# Autodesk Inventor assembly: LF_2
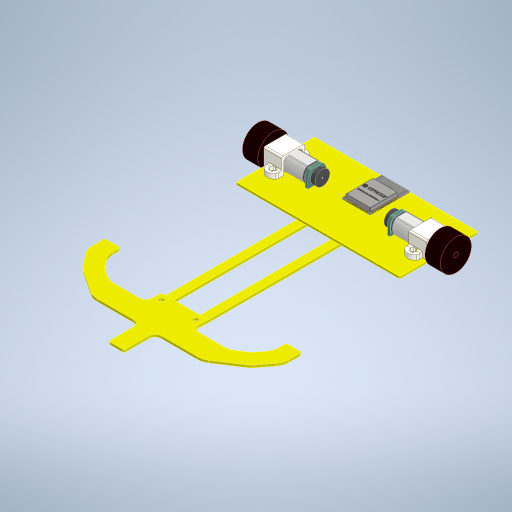
[picture p0: Inventor's stored thumbnail of the model, 512x512]
Saved by Autodesk Inventor 2023 (Build 270158000, 158)
## iProperties
Created: 2024-03-30
Part Number: LF_2
Document SubType Name: Assembly
Designer: Kamil
Author: Kamil
## Documents named in this file (8)
- C:\Users\Kamil\Documents\LineFollower\mechanics\LF_2.iam
- C:\Users\Kamil\Documents\LineFollower\mechanics\belka.ipt
- C:\Users\Kamil\Documents\LineFollower\mechanics\N20 Mini Micro Metall Gear Motor DC 3-6-12V v1.ipt
- C:\Users\Kamil\Documents\LineFollower\mechanics\ESP32-S3-WROOM-1.ipt
- C:\Users\Kamil\Documents\LineFollower\mechanics\ty.ipt
- C:\Users\Kamil\Documents\LineFollower\mechanics\przód.ipt
- C:\Users\Kamil\Documents\LineFollower\mechanics\kolko.ipt
- C:\Users\Kamil\Documents\LineFollower\mechanics\n20_bracket.ipt
## Components (11 placed, 7 different names)
1. belka:1 — Zestawiające:6, Zestawiające:9
2. belka:2 — Zestawiające:7, Zestawiające:8
3. N20 Mini Micro Metall Gear Motor DC 3-6-12V v1:1 — Zestawiające:2, Równoległe:3, Zestawiające:3, Zestawiające:11, Zestawiające:12, Równoległe:10, Zestawiające:17
4. N20 Mini Micro Metall Gear Motor DC 3-6-12V v1:2 — Zestawiające:1, Równoległe:2, Zestawiające:3, Równoległe:4, Zestawiające:10, Zestawiające:13, Równoległe:9, Zestawiające:15
5. ESP32-S3-WROOM-1:1 — Zestawiające:4, Równoległe:5, Równoległe:6
6. ty:1 — Równoległe:1, Zestawiające:1, Zestawiające:2, Równoległe:2, Równoległe:3, Równoległe:4, Zestawiające:4, Równoległe:5, Równoległe:6, Zestawiające:5, Równoległe:7, Równoległe:8, Zestawiające:14, Zestawiające:16
7. przód:1 — Równoległe:1, Zestawiające:5, Równoległe:7, Równoległe:8, Zestawiające:6, Zestawiające:7, Zestawiające:8, Zestawiające:9
8. kolko:1 — Zestawiające:10, Zestawiające:13
9. kolko:2 — Zestawiające:11, Zestawiające:12
10. n20_bracket:1 — Zestawiające:14, Równoległe:9, Zestawiające:15
11. n20_bracket:2 — Zestawiające:16, Równoległe:10, Zestawiające:17
## Relationships (27: Mate 17, Flush 10)
- Równoległe:1 [Flush]: ty:1 ↔ przód:1
- Zestawiające:1 [Mate]: N20 Mini Micro Metall Gear Motor DC 3-6-12V v1:2 ↔ ty:1
- Zestawiające:2 [Mate]: N20 Mini Micro Metall Gear Motor DC 3-6-12V v1:1 ↔ ty:1
- Równoległe:2 [Flush]: N20 Mini Micro Metall Gear Motor DC 3-6-12V v1:2 ↔ ty:1
- Równoległe:3 [Flush]: N20 Mini Micro Metall Gear Motor DC 3-6-12V v1:1 ↔ ty:1
- Zestawiające:3 [Mate]: N20 Mini Micro Metall Gear Motor DC 3-6-12V v1:1 ↔ N20 Mini Micro Metall Gear Motor DC 3-6-12V v1:2
- Równoległe:4 [Flush] (-19 mm): N20 Mini Micro Metall Gear Motor DC 3-6-12V v1:2 ↔ ty:1
- Zestawiające:4 [Mate]: ESP32-S3-WROOM-1:1 ↔ ty:1
- Równoległe:5 [Flush]: ESP32-S3-WROOM-1:1 ↔ ty:1
- Równoległe:6 [Flush] (43.5 mm): ESP32-S3-WROOM-1:1 ↔ ty:1
- Zestawiające:5 [Mate] (-180 mm): ty:1 ↔ przód:1
- Równoległe:7 [Flush] (-10.925 mm): ty:1 ↔ przód:1
- Równoległe:8 [Flush]: ty:1 ↔ przód:1
- Zestawiające:6 [Mate]: belka:1 ↔ przód:1
- Zestawiające:7 [Mate]: belka:2 ↔ przód:1
- Zestawiające:8 [Mate]: belka:2 ↔ przód:1
- Zestawiające:9 [Mate]: belka:1 ↔ przód:1
- Zestawiające:10 [Mate]: N20 Mini Micro Metall Gear Motor DC 3-6-12V v1:2 ↔ kolko:1
- Zestawiające:11 [Mate]: N20 Mini Micro Metall Gear Motor DC 3-6-12V v1:1 ↔ kolko:2
- Zestawiające:12 [Mate] (0.5 mm): N20 Mini Micro Metall Gear Motor DC 3-6-12V v1:1 ↔ kolko:2
- Zestawiające:13 [Mate] (0.5 mm): N20 Mini Micro Metall Gear Motor DC 3-6-12V v1:2 ↔ kolko:1
- Zestawiające:14 [Mate]: ty:1 ↔ n20_bracket:1
- Równoległe:9 [Flush]: N20 Mini Micro Metall Gear Motor DC 3-6-12V v1:2 ↔ n20_bracket:1
- Zestawiające:15 [Mate]: N20 Mini Micro Metall Gear Motor DC 3-6-12V v1:2 ↔ n20_bracket:1
- Zestawiające:16 [Mate]: ty:1 ↔ n20_bracket:2
- Równoległe:10 [Flush]: N20 Mini Micro Metall Gear Motor DC 3-6-12V v1:1 ↔ n20_bracket:2
- Zestawiające:17 [Mate]: N20 Mini Micro Metall Gear Motor DC 3-6-12V v1:1 ↔ n20_bracket:2
